# Autodesk Inventor assembly: 装配-载板
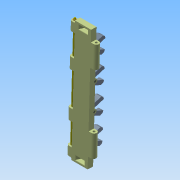
[picture p0: Inventor's stored thumbnail of the model, 180x180]
Saved by Autodesk Inventor 2015 (Build 190159000, 159)
## iProperties
Created: 2017-05-23
Part Number: 装配-载板
Document SubType Name: Assembly
Designer: Administrator
Author: Administrator
## Documents named in this file (8)
- C:\Users\Administrator\Desktop\毕设改\装配-载板.iam
- C:\Users\Administrator\Desktop\毕设改\载板连接销卡环.ipt
- C:\Users\Administrator\Desktop\毕设改\载板.ipt
- C:\Users\Administrator\Desktop\毕设改\载板连接销.ipt
- C:\Users\Administrator\Desktop\毕设改\夹具固定销.ipt
- C:\Users\Administrator\Desktop\毕设改\夹具固定销螺丝.ipt
- C:\Users\Administrator\Desktop\毕设改\夹具右.ipt
- C:\Users\Administrator\Desktop\毕设改\夹具左.ipt
## Components (32 placed, 7 different names)
1. 载板连接销卡环:1 — 配合:1, 相切:1
2. 载板连接销卡环:2 — 配合:2, 相切:2
3. 载板:1 — 插入:1, 相切:1, 相切:2, 插入:2, 插入:3, 表面齐平:1
4. 载板连接销:1 — 插入:1, 配合:1, 配合:2
5. 夹具固定销:1 — 插入:2, 插入:5, 表面齐平:1, 插入:6, 插入:7, 插入:8
6. 夹具固定销螺丝:3 — 插入:6
7. 夹具固定销螺丝:1 — 插入:5
8. 夹具固定销螺丝:2 — 插入:7
9. 夹具固定销螺丝:4 — 插入:8
10. 夹具左:1 — 插入:3, 插入:4
11. 夹具右:1 — 插入:4
12. 夹具固定销:2
13. 夹具固定销螺丝:5
14. 夹具固定销螺丝:6
15. 夹具固定销螺丝:7
16. 夹具固定销螺丝:8
17. 夹具左:2
18. 夹具右:2
19. 夹具固定销:3
20. 夹具固定销螺丝:9
21. 夹具固定销螺丝:10
22. 夹具固定销螺丝:11
23. 夹具固定销螺丝:12
24. 夹具左:3
25. 夹具右:3
26. 夹具固定销:4
27. 夹具固定销螺丝:13
28. 夹具固定销螺丝:14
29. 夹具固定销螺丝:15
30. 夹具固定销螺丝:16
31. 夹具左:4
32. 夹具右:4
## Component patterns: (4 elements, first: 夹具固定销:1 + 夹具固定销螺丝:3 + 夹具固定销螺丝:1 + 夹具固定销螺丝:2 + 夹具固定销螺丝:4 + 夹具左:1 + 夹具右:1)
## Relationships (13: Insert 8, Mate 2, Tangent 2, Flush 1)
- 插入:1 [Insert]: 载板:1 ↔ 载板连接销:1
- 配合:1 [Mate]: 载板连接销卡环:1 ↔ 载板连接销:1
- 相切:1 [Tangent]: 载板连接销卡环:1 ↔ 载板:1
- 配合:2 [Mate]: 载板连接销卡环:2 ↔ 载板连接销:1
- 相切:2 [Tangent]: 载板连接销卡环:2 ↔ 载板:1
- 插入:2 [Insert]: 载板:1 ↔ 夹具固定销:1
- 插入:3 [Insert]: 载板:1 ↔ 夹具左:1
- 插入:4 [Insert]: 夹具左:1 ↔ 夹具右:1
- 插入:5 [Insert]: 夹具固定销:1 ↔ 夹具固定销螺丝:1
- 表面齐平:1 [Flush]: 载板:1 ↔ 夹具固定销:1
- 插入:6 [Insert]: 夹具固定销:1 ↔ 夹具固定销螺丝:3
- 插入:7 [Insert]: 夹具固定销:1 ↔ 夹具固定销螺丝:2
- 插入:8 [Insert]: 夹具固定销:1 ↔ 夹具固定销螺丝:4
